# Autodesk Inventor assembly: ball caster model
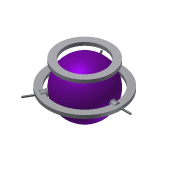
[picture p0: Inventor's stored thumbnail of the model, 180x180]
Saved by Autodesk Inventor 2012 (Build 160160000, 160)
## iProperties
Created: 2011-10-07
Part Number: ball caster model
Document SubType Name: Assembly
Designer: Antonella
Author: Antonella
## Documents named in this file (5)
- C:\Users\Antonella\Documents\GCC Robotics 2012 - Mechanical\Robot 2.0\Ball Caster\ball caster model.iam
- C:\Users\Antonella\Documents\GCC Robotics 2012 - Mechanical\Robot 2.0\Ball Caster\ball model.ipt
- C:\Users\Antonella\Documents\GCC Robotics 2012 - Mechanical\Robot 2.0\Ball Caster\ring_top.ipt
- C:\Users\Antonella\Documents\GCC Robotics 2012 - Mechanical\Robot 2.0\Ball Caster\ring_middle.ipt
- C:\Users\Antonella\Documents\GCC Robotics 2012 - Mechanical\Robot 2.0\Ball Caster\ball_transfer.iam
## Components (6 placed, 4 different names)
1. ball model:1 — Mate:1, Flush:1, Flush:2, Mate:2, Mate:3, Tangent:1, Tangent:2, Tangent:3
2. ring_top:1 — Mate:2, Mate:3
3. ring_middle:1 — Mate:1, Flush:1, Flush:2, Mate:4, Mate:5, Mate:6
4. ball_transfer:1 [sub-assembly] — Mate:4, Tangent:3
5. ball_transfer:2 [sub-assembly] — Mate:6, Tangent:1
6. ball_transfer:3 [sub-assembly] — Mate:5, Tangent:2
## Relationships (11: Mate 6, Tangent 3, Flush 2)
- Mate:1: ball model:1 ↔ ring_middle:1
- Flush:1: ball model:1 ↔ ring_middle:1
- Flush:2: ball model:1 ↔ ring_middle:1
- Mate:2: ball model:1 ↔ ring_top:1
- Mate:3: ball model:1 ↔ ring_top:1
- Mate:4: ring_middle:1 ↔ ball_transfer:1
- Mate:5: ring_middle:1 ↔ ball_transfer:3
- Mate:6: ring_middle:1 ↔ ball_transfer:2
- Tangent:1: ball model:1 ↔ ball_transfer:2
- Tangent:2: ball model:1 ↔ ball_transfer:3
- Tangent:3: ball model:1 ↔ ball_transfer:1
